# Autodesk Inventor assembly: ABD_Slider_Set
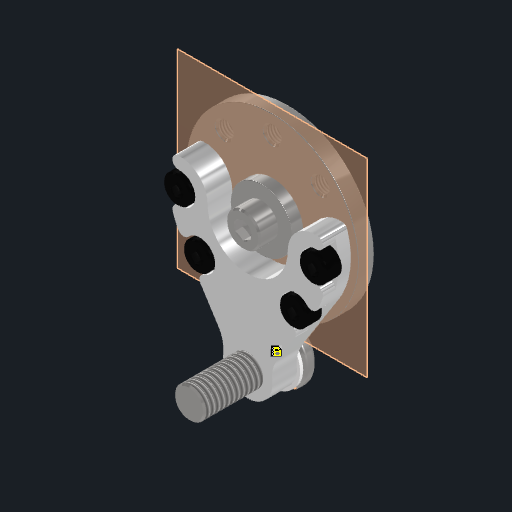
[picture p0: Inventor's stored thumbnail of the model, 512x512]
Saved by Autodesk Inventor 2024.3 (Build 283343000, 343)
## iProperties
Created: 2024-02-15
Part Number: ABD_Slider_Set
Document SubType Name: Assembly
Designer: ASUS
Author: ASUS
## Documents named in this file (7)
- C:\Users\ASUS\Desktop\test\v4_Frame_2025\ABD_Slider_Set_v4.iam
- C:\Users\ASUS\Desktop\test\ROBOTIS(Inventor 2024 ver.)\HORN\64-106Horn.ipt
- C:\Users\ASUS\Desktop\test\v4_Frame_2025\MISUMI\CSH-STN-M3-10.ipt
- C:\Users\ASUS\Desktop\test\v4_Frame_2025\Slider_crank_horn_v4_2025.ipt
- C:\Users\ASUS\Desktop\test\v4_Frame_2025\MISUMI\CSH-ST-M2_5-4.ipt
- C:\Users\ASUS\Desktop\test\v4_Frame_2025\ALI\M5-D6-8mm_Screw.ipt
- C:\Users\ASUS\Desktop\test\v2_Frame\MISUMI\TT-0409-05.ipt
## Components (10 placed, 6 different names)
1. 64-106Horn:1 — 삽입:3, 삽입:4, 메이트:1, 삽입:9
2. CSH-STN-M3-10:1 — 삽입:3
3. Slider_crank_horn_v4_2025:1 — 삽입:4, 메이트:1, 삽입:5, 삽입:6, 삽입:7, 삽입:8, 삽입:11
4. CSH-ST-M2_5-4:1 — 삽입:5
5. CSH-ST-M2_5-4:2 — 삽입:9
6. CSH-ST-M2_5-4:3 — 삽입:6
7. CSH-ST-M2_5-4:4 — 삽입:8
8. CSH-ST-M2_5-4:5 — 삽입:7
9. M5-D6-8mm_Screw:1
10. TT-0409-05:1 — 삽입:11
## Relationships (10: Insert 9, Mate 1)
- 삽입:3 [Insert]: 64-106Horn:1 ↔ CSH-STN-M3-10:1
- 삽입:4 [Insert]: 64-106Horn:1 ↔ Slider_crank_horn_v4_2025:1
- 메이트:1 [Mate]: 64-106Horn:1 ↔ Slider_crank_horn_v4_2025:1
- 삽입:5 [Insert]: Slider_crank_horn_v4_2025:1 ↔ CSH-ST-M2_5-4:1
- 삽입:6 [Insert]: Slider_crank_horn_v4_2025:1 ↔ CSH-ST-M2_5-4:3
- 삽입:7 [Insert]: Slider_crank_horn_v4_2025:1 ↔ CSH-ST-M2_5-4:5
- 삽입:8 [Insert]: Slider_crank_horn_v4_2025:1 ↔ CSH-ST-M2_5-4:4
- 삽입:9 [Insert]: 64-106Horn:1 ↔ CSH-ST-M2_5-4:2
- [Insert]: M5-D6-8mm_Screw:1 ↔ TT-0409-05:1
- 삽입:11 [Insert]: Slider_crank_horn_v4_2025:1 ↔ TT-0409-05:1
